# Autodesk Inventor assembly: Geneva Drive and Frame Assembly
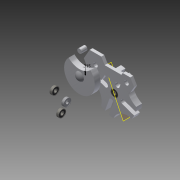
[picture p0: Inventor's stored thumbnail of the model, 180x180]
Saved by Autodesk Inventor 2018 (Build 220112000, 112)
## iProperties
Created: 2018-01-19
Part Number: Geneva Drive and Frame Assembly
Document SubType Name: Assembly
Designer: Rus
Author: Rus
## Documents named in this file (8)
- E:\Libraries\3D Objects\Geneva drive\Mechanical\Attempt 2v2\Geneva Drive and Frame Assembly.iam
- E:\Libraries\3D Objects\Geneva drive\Mechanical\Attempt 2v2\Geneva Drive.ipt
- E:\Libraries\3D Objects\Geneva drive\Mechanical\Attempt 2v2\Geneva Driven.ipt
- E:\Libraries\3D Objects\Geneva drive\Mechanical\Attempt 2v2\Frame.ipt
- E:\Libraries\3D Objects\Geneva drive\Mechanical\Attempt 2v2\608ZZ.iam
- E:\Libraries\3D Objects\Geneva drive\Mechanical\Attempt 2v2\Driver Shaft.ipt
- E:\Libraries\3D Objects\Geneva drive\Mechanical\Attempt 2v2\Driver Input Shaft.ipt
- E:\Libraries\3D Objects\Geneva drive\Mechanical\Attempt 2v2\Driver Shaft Cap.ipt
## Components (10 placed, 7 different names)
1. Geneva Drive:1 — Flush:1, Mate:1, Mate:2
2. Geneva Driven:1 — Insert:1
3. Frame:1
4. 608ZZ:1 [sub-assembly]
5. 608ZZ:2 [sub-assembly]
6. Driver Shaft:1 — Flush:1, Mate:1, Mate:2, Mate:3, Mate:4, Mate:5
7. 608ZZ:3 [sub-assembly]
8. 608ZZ:4 [sub-assembly] — Insert:1
9. Driver Input Shaft:1
10. Driver Shaft Cap:1 — Mate:3, Mate:4, Mate:5
## Relationships (7: Mate 5, Insert 1, Flush 1)
- Insert:1: Geneva Driven:1 ↔ 608ZZ:4
- Flush:1: Geneva Drive:1 ↔ Driver Shaft:1
- Mate:1: Geneva Drive:1 ↔ Driver Shaft:1
- Mate:2: Geneva Drive:1 ↔ Driver Shaft:1
- Mate:3: Driver Shaft:1 ↔ Driver Shaft Cap:1
- Mate:4: Driver Shaft:1 ↔ Driver Shaft Cap:1
- Mate:5: Driver Shaft:1 ↔ Driver Shaft Cap:1
